# Autodesk Inventor assembly: LidAssembly
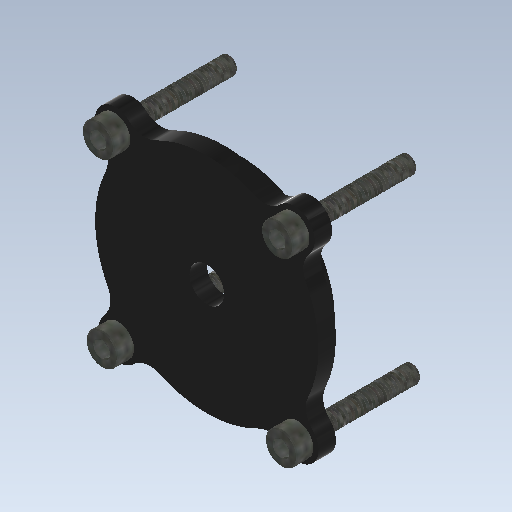
[picture p0: Inventor's stored thumbnail of the model, 512x512]
Saved by Autodesk Inventor 2020.2 (Build 242310000, 310)
## iProperties
Created: 2020-09-03
Part Number: LidAssembly
Document SubType Name: Assembly
Designer: JK
Author: JK
## Documents named in this file (3)
- C:\Users\JK\Documents\Inventor\PeristalticPump\LidAssembly.iam
- C:\Users\JK\Documents\Inventor\PeristalticPump\Lid.ipt
- C:\Users\JK\Documents\Inventor\PeristalticPump\M3x20Bolt.ipt
## Components (5 placed, 2 different names)
1. Lid:1
2. M3x20Bolt:1
3. M3x20Bolt:2
4. M3x20Bolt:3
5. M3x20Bolt:4
## Relationships (8: Mate 5, Flush 3)
- [Mate]: Lid:1 ↔ M3x20Bolt:1
- [Mate]: Lid:1 ↔ M3x20Bolt:2
- [Mate]: Lid:1 ↔ M3x20Bolt:3
- [Mate]: Lid:1 ↔ M3x20Bolt:4
- [Flush]: M3x20Bolt:1 ↔ M3x20Bolt:3
- [Flush]: M3x20Bolt:3 ↔ M3x20Bolt:4
- [Flush]: M3x20Bolt:2 ↔ M3x20Bolt:4
- [Mate]: Lid:1 ↔ M3x20Bolt:2
